# Autodesk Inventor assembly: Turnigy SK8 5045 (IGES V1)
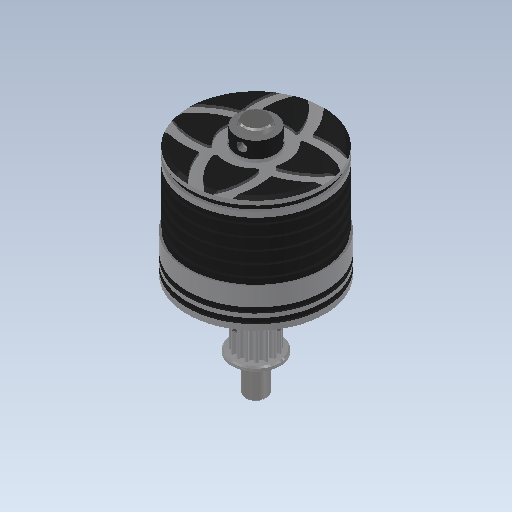
[picture p0: Inventor's stored thumbnail of the model, 512x512]
Saved by Autodesk Inventor 2020.1 (Build 241239000, 239)
## iProperties
Created: 2018-11-25
Part Number: Turnigy SK8 5045 (IGES V1)
Document SubType Name: Assembly
Designer: Petar
Mass: 211.312 g
Surface Area: 494.364 cm^2
Volume: 53.1986 cm^3
Density: 3.97214 g/cm^3
Company: unknown
Title: Turnigy SK8 5045 (IGES V1)
Author: emisnug
## Documents named in this file (9)
- D:\OMG\E-Board\CAD\Inventor\Electric Motor\Turnigy SK8 5045.iam
- D:\OMG\E-Board\CAD\Inventor\Electric Motor\Magnets v9.ipt
- D:\OMG\E-Board\CAD\Inventor\Electric Motor\Can v14.ipt
- D:\OMG\E-Board\CAD\Inventor\Electric Motor\Shaft v2.ipt
- D:\OMG\E-Board\CAD\Inventor\Electric Motor\Stator Core v1.ipt
- D:\OMG\E-Board\CAD\Inventor\Electric Motor\Front Part v5.ipt
- D:\OMG\E-Board\CAD\Inventor\Electric Motor\Bearing (False - Needs Updating) v1.ipt
- D:\OMG\E-Board\CAD\Inventor\Electric Motor\Shuck.ipt
- D:\OMG\E-Board\CAD\Inventor\Mechanical Components\Motor Pulley\Motor Pulley - z16.ipt
## Components (8 placed, 8 different names)
1. Magnets v9:1 — Mate:1, Mate:3, Mate:4, Mate:5, Flush:1
2. Shaft v2:1 — Rigid:1, Rigid:5
3. Stator Core v1:1 — Mate:1, Flush:1
4. Front Part v5:1 — Rigid:6, Insert:1
5. Bearing (False - Needs Updating) v1:1 — Rigid:6
6. Can v14:1 — Mate:3, Mate:4, Mate:5, Rigid:1, Insert:1
7. Motor Pulley - z16:1 — Rigid:7
8. Shuck:1 — Rigid:5, Rigid:7
## Relationships (10: Mate 4, WeldJoint 4, Flush 1, Insert 1)
- Mate:1: Magnets v9:1 ↔ Stator Core v1:1
- Mate:3: Magnets v9:1 ↔ Can v14:1
- Mate:4: Magnets v9:1 ↔ Can v14:1
- Mate:5: Magnets v9:1 ↔ Can v14:1
- Flush:1: Magnets v9:1 ↔ Stator Core v1:1
- Rigid:1 [WeldJoint]: Shaft v2:1 ↔ Can v14:1
- Rigid:5 [WeldJoint]: Shaft v2:1 ↔ Shuck:1
- Rigid:6 [WeldJoint]: Front Part v5:1 ↔ Bearing (False - Needs Updating) v1:1
- Insert:1: Front Part v5:1 ↔ Can v14:1
- Rigid:7 [WeldJoint]: Motor Pulley - z16:1 ↔ Shuck:1
